# Autodesk Inventor assembly: Forearm
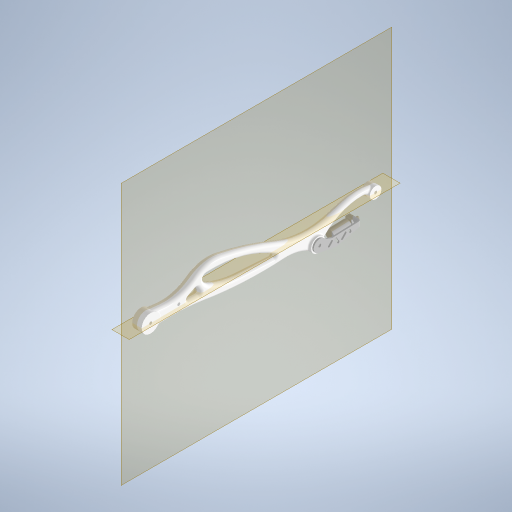
[picture p0: Inventor's stored thumbnail of the model, 512x512]
Saved by Autodesk Inventor 2023 (Build 270158000, 158)
## iProperties
Created: 2023-03-17
Part Number: Forearm
Document SubType Name: Assembly
Designer: valer
Author: valer
## Documents named in this file (4)
- C:\Users\LattePanda\Desktop\str1ker\description\models\src\Forearm.iam
- C:\Users\LattePanda\Desktop\str1ker\parts\Forearm.ipt
- C:\Users\LattePanda\Desktop\str1ker\parts\SolenoidBracket.ipt
- C:\Users\LattePanda\Desktop\str1ker\parts\external\ArmSolenoid.ipt
## Components (3 placed, 3 different names)
1. Forearm:1 — Mate:1, Mate:2, Mate:12, Mate:13, Mate:14
2. SolenoidBracket:1 — Mate:1, Mate:2, Mate:10, Mate:11
3. ArmSolenoid:1 — Mate:10, Mate:11
## Relationships (7: Mate 7)
- Mate:1: Forearm:1 ↔ SolenoidBracket:1
- Mate:2: Forearm:1 ↔ SolenoidBracket:1
- Mate:10: SolenoidBracket:1 ↔ ArmSolenoid:1
- Mate:11: SolenoidBracket:1 ↔ ArmSolenoid:1
- Mate:12: Forearm:1
- Mate:13: Forearm:1
- Mate:14: Forearm:1
